# Autodesk Inventor assembly: Complete Field
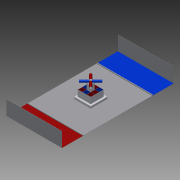
[picture p0: Inventor's stored thumbnail of the model, 180x180]
Saved by Autodesk Inventor 2014 (Build 180170000, 170)
## iProperties
Created: 2014-12-03
Part Number: Complete Field
Document SubType Name: Assembly
Designer: vandenrobots
Author: vandenrobots
## Documents named in this file (3)
- \\DRAFTSERVER\robotics\Green Games\Complete Field.iam
- \\DRAFTSERVER\robotics\Green Games\Field.ipt
- \\DRAFTSERVER\robotics\Green Games\Goals.iam
## Components (2 placed, 2 different names)
1. Field:1 — Mate:1, Flush:1, Mate:2
2. Goals:1 [sub-assembly] — Mate:1, Flush:1, Mate:2
## Relationships (3: Mate 2, Flush 1)
- Mate:1: Field:1 ↔ Goals:1
- Flush:1 (2895.6 mm): Field:1 ↔ Goals:1
- Mate:2 (3962.4 mm): Field:1 ↔ Goals:1
